# Autodesk Inventor assembly: Cube 1x1 V5
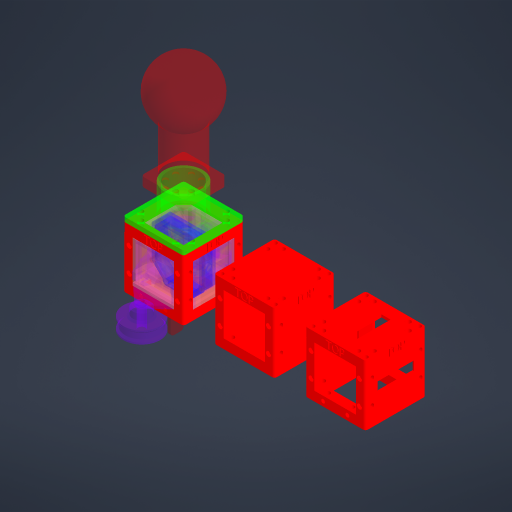
[picture p0: Inventor's stored thumbnail of the model, 512x512]
Saved by Autodesk Inventor 2023.4 (Build 274418000, 418)
## iProperties
Created: 2022-07-25
Part Number: Cube 1x1 V5
Document SubType Name: Assembly
Designer: xSibe
Author: xSibe
## Documents named in this file (58)
- C:\.Laptop\.Work\Projects\Project Protocube\Github\CAD, STL, OBJ Files\1 CAD\Cube 1x1 V5.iam
- C:\.Laptop\.Work\Projects\Project Protocube\1 Autodesk\1 Cubes\Cubes\Cube 1x1 Bottom V5.ipt
- C:\.Laptop\.Work\Projects\Project Protocube\1 Autodesk\1 Cubes\Cubes\Cube 1x1 Top V5.ipt
- C:\.Laptop\.Work\Projects\Project Protocube\1 Autodesk\1 Cubes\Lense\One Inch Lense Holder (V5).ipt
- C:\.Laptop\.Work\Projects\Project Protocube\1 Autodesk\1 Cubes\Lense\Half Inch Lense Holder (V5).ipt
- C:\.Laptop\.Work\Projects\Project Protocube\1 Autodesk\1 Cubes\Laser\Laser Holder (Blue Laser).ipt
- C:\.Laptop\.Work\Projects\Project Protocube\1 Autodesk\1 Cubes\Laser\Laser Holder (Green Laser).ipt
- C:\.Laptop\.Work\Projects\Project Protocube\1 Autodesk\1 Cubes\Sample\Z Axis Sample V1.ipt
- C:\.Laptop\.Work\Projects\Project Protocube\1 Autodesk\1 Cubes\Laser\Laser Holder (Red Laser).ipt
- C:\.Laptop\.Work\Projects\Project Protocube\1 Autodesk\1 Cubes\Objective\Objective Mount.ipt
- C:\.Laptop\.Work\Projects\Project Protocube\1 Autodesk\1 Cubes\Mirror\Mirror Base Vertical.ipt
- C:\.Laptop\.Work\Projects\Project Protocube\1 Autodesk\1 Cubes\Mirror\Mirror Plate Vertical.ipt
- C:\.Laptop\.Work\Projects\Project Protocube\1 Autodesk\1 Cubes\Dichroic\Dichroic Mirror Mount.ipt
- C:\.Laptop\.Work\Projects\Project Protocube\1 Autodesk\1 Cubes\Attachments\Top Mount (SM1).ipt
- C:\.Laptop\.Work\Projects\Project Protocube\1 Autodesk\1 Cubes\Attachments\Flashlight Mount V1.ipt
- C:\.Laptop\.Work\Projects\Project Protocube\1 Autodesk\1 Cubes\Camera\Camera Mount Side.ipt
- C:\.Laptop\.Work\Projects\Project Protocube\1 Autodesk\1 Cubes\Panels\Panel Top 1x1.ipt
- C:\.Laptop\.Work\Projects\Project Protocube\1 Autodesk\1 Cubes\Panels\Panel Side 1x1.ipt
- C:\.Laptop\.Work\Projects\Project Protocube\1 Autodesk\1 Cubes\Panels\Panel Height 1x2.ipt
- C:\.Laptop\.Work\Projects\Project Protocube\1 Autodesk\1 Cubes\Attachments\Tunnel Vertical.ipt
- C:\.Laptop\.Work\Projects\Project Protocube\1 Autodesk\1 Cubes\Attachments\Tunnel Horizontal.ipt
- C:\.Laptop\.Work\Projects\Project Protocube\1 Autodesk\1 Cubes\Panels\Panel Side 1x2.ipt
- C:\.Laptop\.Work\Projects\Project Protocube\1 Autodesk\1 Cubes\Panels\Panel Side 1x3.ipt
- C:\.Laptop\.Work\Projects\Project Protocube\1 Autodesk\1 Cubes\Panels\Panel Side 1x4.ipt
- C:\.Laptop\.Work\Projects\Project Protocube\1 Autodesk\1 Cubes\Panels\Panel Side 1x5.ipt
- C:\.Laptop\.Work\Projects\Project Protocube\1 Autodesk\1 Cubes\Panels\Panel Top 1x2.ipt
- C:\.Laptop\.Work\Projects\Project Protocube\1 Autodesk\1 Cubes\Panels\Panel Top 1x3.ipt
- C:\.Laptop\.Work\Projects\Project Protocube\1 Autodesk\1 Cubes\Panels\Panel Top 1x4.ipt
- C:\.Laptop\.Work\Projects\Project Protocube\1 Autodesk\1 Cubes\Panels\Panel Top 1x5.ipt
- C:\.Laptop\.Work\Projects\Project Protocube\1 Autodesk\1 Cubes\Sample\Z Axis Handle.ipt
- C:\.Laptop\.Work\Projects\Project Protocube\1 Autodesk\1 Cubes\Lense\SM1 Lense Holder (V5).ipt
- C:\.Laptop\.Work\Projects\Project Protocube\1 Autodesk\1 Cubes\Mirror\Mirror Base Horizontal.ipt
- C:\.Laptop\.Work\Projects\Project Protocube\1 Autodesk\1 Cubes\Mirror\Mirror Plate Horizontal.ipt
- C:\.Laptop\.Work\Projects\Project Protocube\1 Autodesk\1 Cubes\Tools\Baseplate V5 Press.ipt
- C:\.Laptop\.Work\Projects\Project Protocube\1 Autodesk\1 Cubes\Attachments\Cover Top (Full).ipt
- C:\.Laptop\.Work\Projects\Project Protocube\1 Autodesk\1 Cubes\Tools\Laser Alignment Tool V1.ipt
- C:\.Laptop\.Work\Projects\Project Protocube\1 Autodesk\1 Cubes\Filter\Filter Mount (SM05).ipt
- C:\.Laptop\.Work\Projects\Project Protocube\1 Autodesk\1 Cubes\Filter\Filter Mount (SM1).ipt
- C:\.Laptop\.Work\Projects\Project Protocube\1 Autodesk\1 Cubes\Covers\Cover Side (Normal).ipt
- C:\.Laptop\.Work\Projects\Project Protocube\1 Autodesk\1 Cubes\Covers\Cover Top (Normal) Proto.ipt
- C:\.Laptop\.Work\Projects\Project Protocube\1 Autodesk\1 Cubes\Covers\Cover Side (Slotted).ipt
- C:\.Laptop\.Work\Projects\Project Protocube\1 Autodesk\1 Cubes\Covers\Cover Top (Slotted) Proto.ipt
- C:\.Laptop\.Work\Projects\Project Protocube\1 Autodesk\1 Cubes\Cubes\Cube 1x1 Top V5 Closed.ipt
- C:\.Laptop\.Work\Projects\Project Protocube\1 Autodesk\1 Cubes\Cubes\Cube 1x1 Bottom V5 Closed.ipt
- C:\.Laptop\.Work\Projects\Project Protocube\1 Autodesk\1 Cubes\Cubes\Cube 1x1 Bottom V5 Closed Slotted.ipt
- C:\.Laptop\.Work\Projects\Project Protocube\1 Autodesk\1 Cubes\Cubes\Cube 1x1 Top V5 Closed Slotted.ipt
- C:\.Laptop\.Work\Projects\Project Protocube\1 Autodesk\1 Cubes\Lense\Half Inch Lense Holder Cover (V5).ipt
- C:\.Laptop\.Work\Projects\Project Protocube\1 Autodesk\1 Cubes\Lense\One Inch Lense Holder Cover (V5).ipt
- C:\.Laptop\.Work\Projects\Project Protocube\1 Autodesk\1 Cubes\Tools\Laser Alignment Tool V2.ipt
- C:\.Laptop\.Work\Projects\Project Protocube\1 Autodesk\1 Cubes\Lense\SM05 Lense Holder (V5).ipt
- C:\.Laptop\.Work\Projects\Project Protocube\1 Autodesk\1 Cubes\Laser\Laser Switch.ipt
- C:\.Laptop\.Work\Projects\Project Protocube\1 Autodesk\1 Cubes\Laser\Laser Holder (USB Laser).ipt
- C:\.Laptop\.Work\Projects\Project Protocube\1 Autodesk\1 Cubes\XYZ Stage\Z Stage Body V5.ipt
- C:\.Laptop\.Work\Projects\Project Protocube\1 Autodesk\1 Cubes\Attachments\Top Mount (SM05).ipt
- C:\.Laptop\.Work\Projects\Project Protocube\1 Autodesk\1 Cubes\Tools\Cube 1x1 V5 Bot Press.ipt
- C:\.Laptop\.Work\Projects\Project Protocube\1 Autodesk\1 Cubes\Tools\Cube 1x1 V5 Top Press.ipt
- C:\.Laptop\.Work\Projects\Project Protocube\1 Autodesk\1 Cubes\Filter\Filter Adapter (SM1).ipt
- C:\.Laptop\.Work\Projects\Project Protocube\1 Autodesk\1 Cubes\Filter\Filter Adapter (SM05).ipt
## Components (58 placed, 57 different names)
1. Cube 1x1 Top V5:1 — Mate:1, Mate:2, Mate:3, Mate:4, Mate:5, Mate:6, Mate:40, Flush:23, Flush:24, Mate:60, Mate:61, Mate:62, Mate:63, Mate:64, Mate:65
2. Cube 1x1 Bottom V5:1 — Mate:1, Mate:2, Mate:3, Mate:9, Mate:10, Mate:11, Mate:39, Flush:21
3. Cube 1x1 Top V5 Closed:1 — Mate:40, Flush:23, Flush:24, Mate:41, Mate:42, Mate:43
4. Cube 1x1 Bottom V5 Closed:1 — Mate:41, Mate:42, Mate:43, Mate:54, Mate:55, Mate:56
5. Cube 1x1 Top V5 Closed Slotted:1 — Mate:51, Mate:52, Mate:53
6. Cube 1x1 Bottom V5 Closed Slotted:1 — Mate:51, Mate:52, Mate:53, Mate:54, Mate:55, Mate:56
7. Z Axis Handle:1 — Mate:34, Mate:35
8. Z Axis Handle:2 — Mate:36, Mate:37
9. Laser Alignment Tool V1:1 — Flush:18
10. Laser Alignment Tool V2:1
11. Baseplate V5 Press:1 — Flush:15
12. Cube 1x1 V5 Bot Press:1
13. Cube 1x1 V5 Top Press:1
14. Laser Switch:1
15. Z Stage Body V5:1
16. Half Inch Lense Holder Cover (V5):1
17. One Inch Lense Holder Cover (V5):1
18. Half Inch Lense Holder (V5):1
19. One Inch Lense Holder (V5):1 — Flush:1
20. Laser Holder (Red Laser):1
21. Laser Holder (Green Laser):1
22. Laser Holder (Blue Laser):1
23. Laser Holder (USB Laser):1
24. SM05 Lense Holder (V5):1
25. SM1 Lense Holder (V5):1
26. Filter Mount (SM05):1 — Flush:19
27. Filter Mount (SM1):1
28. Tunnel Vertical:1 — Flush:10
29. Tunnel Horizontal:1 — Flush:11
30. Mirror Base Vertical:1 — Flush:5
31. Mirror Plate Vertical:1
32. Mirror Base Horizontal:1 — Flush:12, Flush:14
33. Mirror Plate Horizontal:1 — Mate:38, Flush:13, Flush:14
34. Z Axis Sample V1:1 — Flush:2, Mate:34, Mate:35, Mate:36, Mate:37
35. Dichroic Mirror Mount:1 — Flush:6
36. Camera Mount Side:1 — Flush:7
37. Objective Mount:1 — Flush:4
38. Filter Adapter (SM1):1
39. Filter Adapter (SM05):1
40. Top Mount (SM1):1 — Mate:4, Mate:5, Mate:6
41. Top Mount (SM05):1 — Mate:60, Mate:61, Mate:62
42. Flashlight Mount V1:1 — Mate:63, Mate:64, Mate:65
43. Cover Top (Full):1 — Flush:17
44. Cover Side (Normal):1 — Flush:20, Mate:39, Flush:21
45. Cover Side (Slotted):1
46. Cover Top (Normal) Proto:1 — Flush:22
47. Cover Top (Slotted) Proto:1
48. Panel Height 1x2:1 — Mate:9, Mate:10, Mate:11
49. Panel Top 1x1:1 — Flush:8, Mate:30, Mate:31
50. Panel Top 1x2:1 — Mate:21, Mate:22, Mate:29
51. Panel Top 1x3:1 — Mate:21, Mate:22, Mate:23, Mate:24, Mate:28, Mate:30
52. Panel Top 1x4:1 — Mate:23, Mate:24, Mate:25, Mate:26, Mate:27, Mate:29, Mate:31
53. Panel Top 1x5:1 — Mate:25, Mate:26, Mate:27, Mate:28
54. Panel Side 1x1:1 — Flush:9, Mate:32, Mate:33
55. Panel Side 1x2:1 — Mate:12, Mate:13, Mate:20
56. Panel Side 1x3:1 — Mate:12, Mate:13, Mate:14, Mate:15, Mate:19
57. Panel Side 1x4:1 — Mate:14, Mate:15, Mate:16, Mate:17, Mate:18, Mate:20, Mate:32
58. Panel Side 1x5:1 — Mate:16, Mate:17, Mate:18, Mate:19, Mate:33
## Relationships (75: Mate 53, Flush 22)
- Mate:1: Cube 1x1 Top V5:1 ↔ Cube 1x1 Bottom V5:1
- Mate:2: Cube 1x1 Top V5:1 ↔ Cube 1x1 Bottom V5:1
- Mate:3: Cube 1x1 Top V5:1 ↔ Cube 1x1 Bottom V5:1
- Flush:1: One Inch Lense Holder (V5):1
- Flush:2: Z Axis Sample V1:1
- Flush:4: Objective Mount:1
- Flush:5: Mirror Base Vertical:1
- Flush:6: Dichroic Mirror Mount:1
- Mate:4: Cube 1x1 Top V5:1 ↔ Top Mount (SM1):1
- Mate:5: Cube 1x1 Top V5:1 ↔ Top Mount (SM1):1
- Mate:6: Cube 1x1 Top V5:1 ↔ Top Mount (SM1):1
- Flush:7: Camera Mount Side:1
- Flush:8: Panel Top 1x1:1
- Flush:9: Panel Side 1x1:1
- Mate:9: Cube 1x1 Bottom V5:1 ↔ Panel Height 1x2:1
- Mate:10: Cube 1x1 Bottom V5:1 ↔ Panel Height 1x2:1
- Mate:11: Cube 1x1 Bottom V5:1 ↔ Panel Height 1x2:1
- Flush:10: Tunnel Vertical:1
- Flush:11: Tunnel Horizontal:1
- Mate:12: Panel Side 1x2:1 ↔ Panel Side 1x3:1
- Mate:13: Panel Side 1x2:1 ↔ Panel Side 1x3:1
- Mate:14: Panel Side 1x3:1 ↔ Panel Side 1x4:1
- Mate:15: Panel Side 1x3:1 ↔ Panel Side 1x4:1
- Mate:16: Panel Side 1x4:1 ↔ Panel Side 1x5:1
- Mate:17: Panel Side 1x4:1 ↔ Panel Side 1x5:1
- Mate:18: Panel Side 1x4:1 ↔ Panel Side 1x5:1
- Mate:19: Panel Side 1x3:1 ↔ Panel Side 1x5:1
- Mate:20: Panel Side 1x2:1 ↔ Panel Side 1x4:1
- Mate:21: Panel Top 1x2:1 ↔ Panel Top 1x3:1
- Mate:22: Panel Top 1x2:1 ↔ Panel Top 1x3:1
- Mate:23: Panel Top 1x3:1 ↔ Panel Top 1x4:1
- Mate:24: Panel Top 1x3:1 ↔ Panel Top 1x4:1
- Mate:25: Panel Top 1x4:1 ↔ Panel Top 1x5:1
- Mate:26: Panel Top 1x4:1 ↔ Panel Top 1x5:1
- Mate:27: Panel Top 1x4:1 ↔ Panel Top 1x5:1
- Mate:28: Panel Top 1x3:1 ↔ Panel Top 1x5:1
- Mate:29: Panel Top 1x2:1 ↔ Panel Top 1x4:1
- Mate:30: Panel Top 1x1:1 ↔ Panel Top 1x3:1
- Mate:31: Panel Top 1x1:1 ↔ Panel Top 1x4:1
- Mate:32: Panel Side 1x1:1 ↔ Panel Side 1x4:1
- Mate:33: Panel Side 1x1:1 ↔ Panel Side 1x5:1
- Mate:34: Z Axis Handle:1 ↔ Z Axis Sample V1:1
- Mate:35: Z Axis Handle:1 ↔ Z Axis Sample V1:1
- Mate:36: Z Axis Handle:2 ↔ Z Axis Sample V1:1
- Mate:37: Z Axis Handle:2 ↔ Z Axis Sample V1:1
- Flush:12: Mirror Base Horizontal:1
- Mate:38: Mirror Plate Horizontal:1
- Flush:13: Mirror Plate Horizontal:1
- Flush:14: Mirror Base Horizontal:1 ↔ Mirror Plate Horizontal:1
- Flush:15: Baseplate V5 Press:1
- Flush:17: Cover Top (Full):1
- Flush:18: Laser Alignment Tool V1:1
- Flush:19: Filter Mount (SM05):1
- Flush:20: Cover Side (Normal):1
- Mate:39: Cube 1x1 Bottom V5:1 ↔ Cover Side (Normal):1
- Flush:21: Cube 1x1 Bottom V5:1 ↔ Cover Side (Normal):1
- Flush:22: Cover Top (Normal) Proto:1
- Mate:40 (25 mm): Cube 1x1 Top V5:1 ↔ Cube 1x1 Top V5 Closed:1
- Flush:23: Cube 1x1 Top V5:1 ↔ Cube 1x1 Top V5 Closed:1
- Flush:24: Cube 1x1 Top V5:1 ↔ Cube 1x1 Top V5 Closed:1
- Mate:41: Cube 1x1 Top V5 Closed:1 ↔ Cube 1x1 Bottom V5 Closed:1
- Mate:42: Cube 1x1 Top V5 Closed:1 ↔ Cube 1x1 Bottom V5 Closed:1
- Mate:43: Cube 1x1 Top V5 Closed:1 ↔ Cube 1x1 Bottom V5 Closed:1
- Mate:51: Cube 1x1 Top V5 Closed Slotted:1 ↔ Cube 1x1 Bottom V5 Closed Slotted:1
- Mate:52: Cube 1x1 Top V5 Closed Slotted:1 ↔ Cube 1x1 Bottom V5 Closed Slotted:1
- Mate:53: Cube 1x1 Top V5 Closed Slotted:1 ↔ Cube 1x1 Bottom V5 Closed Slotted:1
- Mate:54 (25 mm): Cube 1x1 Bottom V5 Closed:1 ↔ Cube 1x1 Bottom V5 Closed Slotted:1
- Mate:55: Cube 1x1 Bottom V5 Closed:1 ↔ Cube 1x1 Bottom V5 Closed Slotted:1
- Mate:56: Cube 1x1 Bottom V5 Closed:1 ↔ Cube 1x1 Bottom V5 Closed Slotted:1
- Mate:60: Cube 1x1 Top V5:1 ↔ Top Mount (SM05):1
- Mate:61: Cube 1x1 Top V5:1 ↔ Top Mount (SM05):1
- Mate:62: Cube 1x1 Top V5:1 ↔ Top Mount (SM05):1
- Mate:63: Cube 1x1 Top V5:1 ↔ Flashlight Mount V1:1
- Mate:64: Cube 1x1 Top V5:1 ↔ Flashlight Mount V1:1
- Mate:65: Cube 1x1 Top V5:1 ↔ Flashlight Mount V1:1
